# Autodesk Inventor assembly: Tire_MIR2
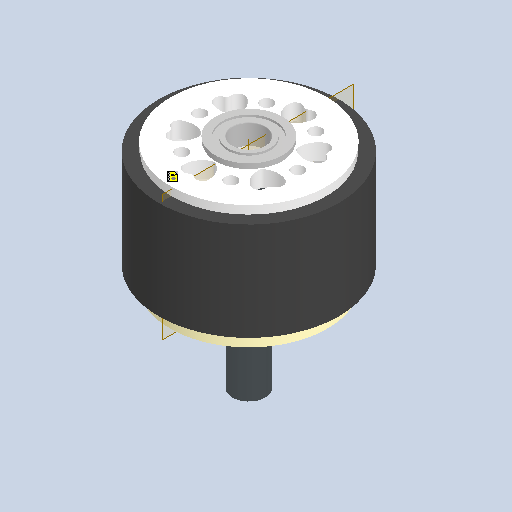
[picture p0: Inventor's stored thumbnail of the model, 512x512]
Saved by Autodesk Inventor 2022 (Build 260153000, 153)
## iProperties
Created: 2021-09-23
Part Number: Tire_MIR2
Document SubType Name: Assembly
Designer: shiokaze
Mass: 6.37362 g
Surface Area: 59.289 cm^2
Volume: 3.61915 cm^3
Author: shiok
## Documents named in this file (7)
- C:\Users\Yazawa\Documents\GitHub\murakumo\inventor\Tire_MIR2.iam
- C:\Users\Yazawa\Documents\GitHub\murakumo\inventor\wheel_MIR2.ipt
- C:\Users\Yazawa\Documents\GitHub\murakumo\inventor\wheelcap_MIR2.ipt
- C:\Users\Yazawa\Documents\GitHub\murakumo\inventor\Tire_MIR2.ipt
- C:\Users\Yazawa\Documents\GitHub\murakumo\inventor\spergear_MIR2.ipt
- C:\Users\Yazawa\Documents\GitHub\murakumo\inventor\FL674ZZ_MIR2.ipt
- C:\Users\Yazawa\Documents\GitHub\murakumo\inventor\shaft_MIR2.ipt
## Components (8 placed, 6 different names)
1. wheel_MIR2:1 — 挿入:1, 挿入:2, 挿入:3, メイト:1, メイト:5, メイト:4
2. wheelcap_MIR2:1 — 挿入:1, メイト:7, メイト:6
3. Tire_MIR2:1 — 挿入:2
4. spergear_MIR2:1 — 挿入:3, メイト:1, メイト:3, メイト:2
5. FL674ZZ_MIR2:1 — メイト:3, メイト:2
6. FL674ZZ_MIR2:2 — メイト:5, メイト:4
7. FL674ZZ_MIR2:3 — メイト:7, メイト:6, 挿入:4, フラッシュ:9
8. shaft_MIR2:1 — 挿入:4, フラッシュ:9
## Relationships (12: Mate 7, Insert 4, Flush 1)
- 挿入:1 [Insert]: wheel_MIR2:1 ↔ wheelcap_MIR2:1
- 挿入:2 [Insert]: wheel_MIR2:1 ↔ Tire_MIR2:1
- 挿入:3 [Insert]: wheel_MIR2:1 ↔ spergear_MIR2:1
- メイト:1 [Mate]: wheel_MIR2:1 ↔ spergear_MIR2:1
- メイト:3 [Mate]: spergear_MIR2:1 ↔ FL674ZZ_MIR2:1
- メイト:2 [Mate]: spergear_MIR2:1 ↔ FL674ZZ_MIR2:1
- メイト:5 [Mate]: wheel_MIR2:1 ↔ FL674ZZ_MIR2:2
- メイト:4 [Mate]: wheel_MIR2:1 ↔ FL674ZZ_MIR2:2
- メイト:7 [Mate]: wheelcap_MIR2:1 ↔ FL674ZZ_MIR2:3
- メイト:6 [Mate]: wheelcap_MIR2:1 ↔ FL674ZZ_MIR2:3
- 挿入:4 [Insert]: FL674ZZ_MIR2:3 ↔ shaft_MIR2:1
- フラッシュ:9 [Flush]: FL674ZZ_MIR2:3 ↔ shaft_MIR2:1
